# Autodesk Inventor assembly: Test for new Cast Assembly
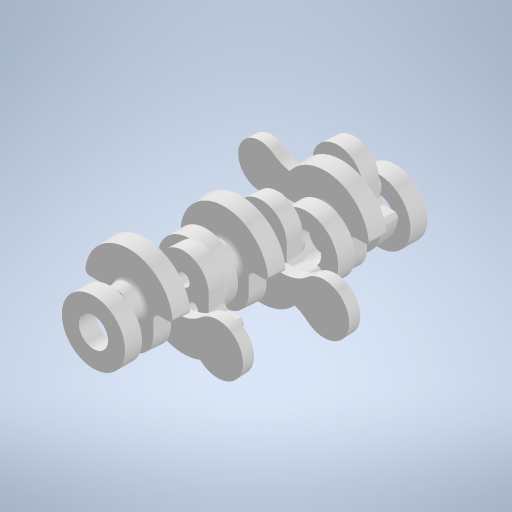
[picture p0: Inventor's stored thumbnail of the model, 512x512]
Saved by Autodesk Inventor 2023 (Build 270158000, 158)
## iProperties
Created: 2022-12-31
Part Number: Test for new Cast Assembly
Document SubType Name: Assembly
Designer: tommy
Author: tommy
## Documents named in this file (4)
- C:\Users\tgr41\OneDrive\Documents\Repositories\Steam-Engine\1.5x1 Inch 3 Cylidner\2 Inch V3\Test for new Cast Assembly.iam
- C:\Users\tgr41\OneDrive\Documents\Repositories\Steam-Engine\1.5x1 Inch 3 Cylidner\2 Inch V3\Connecting Rod Cast Image.ipt
- C:\Users\tgr41\OneDrive\Documents\Repositories\Steam-Engine\1.5x1 Inch 3 Cylidner\2 Inch V3\Crank on Crankshaft.ipt
- C:\Users\tgr41\OneDrive\Documents\Repositories\Steam-Engine\1.5x1 Inch 3 Cylidner\2 Inch V3\CrankShaft Main Bearing.ipt
## Components (13 placed, 3 different names)
1. Connecting Rod Cast Image:1 — Mate:1, Mate:2
2. Crank on Crankshaft:1 — Mate:2, Mate:3
3. Crank on Crankshaft:2 — Mate:1, Mate:10
4. CrankShaft Main Bearing:2 — Mate:3, Mate:11
5. Connecting Rod Cast Image:2
6. Crank on Crankshaft:3
7. Crank on Crankshaft:4 — Mate:11
8. CrankShaft Main Bearing:3
9. Connecting Rod Cast Image:3
10. Crank on Crankshaft:5
11. Crank on Crankshaft:6 — Mate:12
12. CrankShaft Main Bearing:4 — Mate:10
13. CrankShaft Main Bearing:5 — Mate:12
## Relationships (12: Mate 12)
- Mate:1: Connecting Rod Cast Image:1 ↔ Crank on Crankshaft:2
- Mate:2: Connecting Rod Cast Image:1 ↔ Crank on Crankshaft:1
- Mate:3: Crank on Crankshaft:1 ↔ CrankShaft Main Bearing:2
- [Mate]: Connecting Rod Cast Image:2 ↔ Crank on Crankshaft:4
- [Mate]: Connecting Rod Cast Image:2 ↔ Crank on Crankshaft:3
- [Mate]: Crank on Crankshaft:3 ↔ CrankShaft Main Bearing:3
- [Mate]: Connecting Rod Cast Image:3 ↔ Crank on Crankshaft:6
- [Mate]: Connecting Rod Cast Image:3 ↔ Crank on Crankshaft:5
- [Mate]: Crank on Crankshaft:5 ↔ CrankShaft Main Bearing:4
- Mate:10: Crank on Crankshaft:2 ↔ CrankShaft Main Bearing:4
- Mate:11: CrankShaft Main Bearing:2 ↔ Crank on Crankshaft:4
- Mate:12: Crank on Crankshaft:6 ↔ CrankShaft Main Bearing:5
## Named parameters: d4_d0 = 0 mm, d5_d1 = 0 mm, d6_d2 = 0 mm, d7_d0 = 0 mm, d8_d1 = 0 mm, d9_d2 = 0 mm
